# Autodesk Inventor assembly: WheelAssembly_v8_MIR
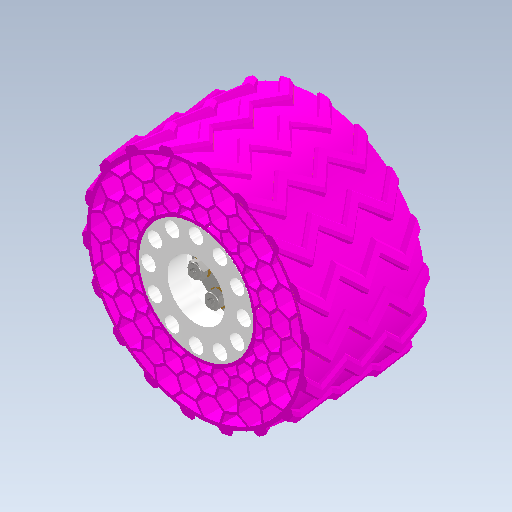
[picture p0: Inventor's stored thumbnail of the model, 512x512]
Saved by Autodesk Inventor 2023 (Build 270158000, 158)
## iProperties
Created: 2023-04-06
Part Number: WheelAssembly_v8_MIR
Document SubType Name: Assembly
Designer: Dave
Mass: 719.998 g
Surface Area: 4242.43 cm^2
Volume: 481.212 cm^3
Density: 1.49622 g/cm^3
Author: asach
## Documents named in this file (7)
- C:\Users\Dave\Documents\GitHub\BehrendURCMechanical\CAD\Chassis V3\Wheel\WheelAssembly_v8_MIR.iam
- C:\Users\Dave\Documents\GitHub\BehrendURCMechanical\CAD\Chassis V3\Wheel\Tire_v8_MIR.ipt
- C:\Users\Dave\Documents\GitHub\BehrendURCMechanical\CAD\Chassis V3\Wheel\ThickWheelPlate_v8_MIR.ipt
- C:\Users\Dave\Documents\GitHub\BehrendURCMechanical\CAD\Chassis V3\Wheel\Washer_MIR.ipt
- C:\Users\Dave\Documents\GitHub\BehrendURCMechanical\CAD\Chassis V3\Wheel\WheelPlateBolt_1inch_MIR.ipt
- C:\Users\Dave\Documents\GitHub\BehrendURCMechanical\CAD\Chassis V3\Wheel\WheelPlateNut_MIR.ipt
- C:\Users\Dave\Documents\GitHub\BehrendURCMechanical\CAD\Chassis V3\Wheel\HubCap_v7_MIR.ipt
## Components (53 placed, 6 different names)
1. Tire_v8_MIR:1 — Mate:3, Mate:2, Mate:1, Mate:6, Mate:5, Mate:4, Mate:7, Mate:16, Mate:19
2. ThickWheelPlate_v8_MIR:1 — Mate:3, Mate:2, Mate:1, Mate:10, Mate:15
3. ThickWheelPlate_v8_MIR:2 — Mate:6, Mate:5, Mate:4, Mate:12, Mate:14, Mate:18
4. HubCap_v7_MIR:1 — Mate:16, Mate:15, Mate:17
5. HubCap_v7_MIR:2 — Mate:20, Mate:19, Mate:18
6. Washer_MIR:1 — Mate:12, Mate:11, Mate:20
7. Washer_MIR:2 — Mate:10, Mate:9, Mate:8
8. WheelPlateBolt_1inch_MIR:1 — Mate:7, Mate:9, Mate:8, Mate:11, Mate:13
9. WheelPlateNut_MIR:1 — Mate:14, Mate:13
10. Washer_MIR:3
11. Washer_MIR:4
12. WheelPlateBolt_1inch_MIR:2
13. WheelPlateNut_MIR:2
14. Washer_MIR:5
15. Washer_MIR:6
16. WheelPlateBolt_1inch_MIR:3 — Mate:17
17. WheelPlateNut_MIR:3
18. Washer_MIR:7
19. Washer_MIR:8
20. WheelPlateBolt_1inch_MIR:4
21. WheelPlateNut_MIR:4
22. Washer_MIR:9
23. Washer_MIR:10
24. WheelPlateBolt_1inch_MIR:5
25. WheelPlateNut_MIR:5
26. Washer_MIR:11
27. Washer_MIR:12
28. WheelPlateBolt_1inch_MIR:6
29. WheelPlateNut_MIR:6
30. Washer_MIR:13
31. Washer_MIR:14
32. WheelPlateBolt_1inch_MIR:7
33. WheelPlateNut_MIR:7
34. Washer_MIR:15
35. Washer_MIR:16
36. WheelPlateBolt_1inch_MIR:8
37. WheelPlateNut_MIR:8
38. Washer_MIR:17
39. Washer_MIR:18
40. WheelPlateBolt_1inch_MIR:9
41. WheelPlateNut_MIR:9
42. Washer_MIR:19
43. Washer_MIR:20
44. WheelPlateBolt_1inch_MIR:10
45. WheelPlateNut_MIR:10
46. Washer_MIR:21
47. Washer_MIR:22
48. WheelPlateBolt_1inch_MIR:11
49. WheelPlateNut_MIR:11
50. Washer_MIR:23
51. Washer_MIR:24
52. WheelPlateBolt_1inch_MIR:12
53. WheelPlateNut_MIR:12
## Component patterns: (12 elements, first: Washer_MIR:1 + Washer_MIR:2 + WheelPlateBolt_1inch_MIR:1 + WheelPlateNut_MIR:1)
## Relationships (20: Mate 20)
- Mate:3: Tire_v8_MIR:1 ↔ ThickWheelPlate_v8_MIR:1
- Mate:2: Tire_v8_MIR:1 ↔ ThickWheelPlate_v8_MIR:1
- Mate:1: Tire_v8_MIR:1 ↔ ThickWheelPlate_v8_MIR:1
- Mate:6: Tire_v8_MIR:1 ↔ ThickWheelPlate_v8_MIR:2
- Mate:5: Tire_v8_MIR:1 ↔ ThickWheelPlate_v8_MIR:2
- Mate:4: Tire_v8_MIR:1 ↔ ThickWheelPlate_v8_MIR:2
- Mate:7: Tire_v8_MIR:1 ↔ WheelPlateBolt_1inch_MIR:1
- Mate:10: ThickWheelPlate_v8_MIR:1 ↔ Washer_MIR:2
- Mate:9: Washer_MIR:2 ↔ WheelPlateBolt_1inch_MIR:1
- Mate:8: Washer_MIR:2 ↔ WheelPlateBolt_1inch_MIR:1
- Mate:12: ThickWheelPlate_v8_MIR:2 ↔ Washer_MIR:1
- Mate:11: Washer_MIR:1 ↔ WheelPlateBolt_1inch_MIR:1
- Mate:14: ThickWheelPlate_v8_MIR:2 ↔ WheelPlateNut_MIR:1
- Mate:13: WheelPlateBolt_1inch_MIR:1 ↔ WheelPlateNut_MIR:1
- Mate:16: Tire_v8_MIR:1 ↔ HubCap_v7_MIR:1
- Mate:15: ThickWheelPlate_v8_MIR:1 ↔ HubCap_v7_MIR:1
- Mate:20: HubCap_v7_MIR:2 ↔ Washer_MIR:1
- Mate:19: Tire_v8_MIR:1 ↔ HubCap_v7_MIR:2
- Mate:18: ThickWheelPlate_v8_MIR:2 ↔ HubCap_v7_MIR:2
- Mate:17: HubCap_v7_MIR:1 ↔ WheelPlateBolt_1inch_MIR:3
